# Autodesk Inventor assembly: volledige behuizing
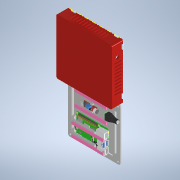
[picture p0: Inventor's stored thumbnail of the model, 180x180]
Saved by Autodesk Inventor 2021 (Build 250183000, 183)
## iProperties
Created: 2023-10-02
Part Number: volledige behuizing
Document SubType Name: Assembly
Designer: Elias
Author: Elias
## Documents named in this file (11)
- D:\Hoge school ICT\2.0 Project experience 2.1\Tekeningen\volledige behuizing.iam
- D:\Hoge school ICT\2.0 Project experience 2.1\Tekeningen\Led behuizing.ipt
- D:\Hoge school ICT\2.0 Project experience 2.1\Tekeningen\Led deksel.ipt
- D:\Hoge school ICT\2.0 Project experience 2.1\Tekeningen\Raspberry Pi 4 Model B.iam
- D:\Hoge school ICT\2.0 Project experience 2.1\Tekeningen\zweef.ipt
- D:\Hoge school ICT\2.0 Project experience 2.1\Tekeningen\geluid sensor.ipt
- D:\Hoge school ICT\2.0 Project experience 2.1\Tekeningen\zweef-01.ipt
- D:\Hoge school ICT\2.0 Project experience 2.1\Tekeningen\koppelstuk.ipt
- D:\Hoge school ICT\2.0 Project experience 2.1\Tekeningen\dc-barrel-jack-adapter-female-with-screw-terminals-1.snapshot.2\dc-barrel-jack-adapter-female.iam
- D:\Hoge school ICT\2.0 Project experience 2.1\Tekeningen\Microphone Module.ipt
- D:\Hoge school ICT\2.0 Project experience 2.1\Tekeningen\ledstrip.ipt
## Components (15 placed, 10 different names)
1. Led behuizing:1 — Mate:2, Mate:3, Mate:4, Flush:6, Mate:9, Flush:7, Mate:12, Flush:10, Tangent:1, Mate:14
2. Led deksel:1 — Mate:2, Mate:3, Insert:1, Insert:2, Mate:4, Flush:1, Mate:5, Flush:2, Mate:6, Mate:8, Flush:4, Flush:5, Tangent:2, Mate:15, Mate:18, Mate:19, Flush:11, Flush:12
3. Raspberry Pi 4 Model B:1 [sub-assembly] — Insert:1, Insert:2
4. zweef:1 — Flush:1, Mate:5, Flush:2, Mate:7, Flush:3, Mate:17
5. geluid sensor:1 — Mate:8, Flush:4, Flush:5
6. zweef-01:1 — Mate:6, Mate:7, Flush:3, Mate:16
7. Led behuizing:2 — Flush:6, Mate:9, Flush:7, Mate:10, Mate:11, Flush:8, Mate:13, Flush:9
8. koppelstuk:1 — Mate:10, Mate:11, Flush:8
9. koppelstuk:2 — Mate:12, Mate:13, Flush:9
10. dc-barrel-jack-adapter-female:1 [sub-assembly] — Flush:10, Tangent:1, Mate:14
11. Microphone Module:2 — Tangent:2, Mate:15
12. ledstrip:1 — Mate:18, Flush:11, Flush:12, Flush:13, Flush:14, Mate:20
13. ledstrip:2 — Mate:19, Flush:13, Mate:20, Mate:21
14. ledstrip:3 — Mate:16, Flush:14, Mate:21, Mate:22, Flush:15
15. ledstrip:4 — Mate:17, Flush:15, Mate:22
## Relationships (40: Mate 21, Flush 15, Insert 2, Tangent 2)
- Mate:2: Led behuizing:1 ↔ Led deksel:1
- Mate:3: Led behuizing:1 ↔ Led deksel:1
- Insert:1: Led deksel:1 ↔ Raspberry Pi 4 Model B:1
- Insert:2: Led deksel:1 ↔ Raspberry Pi 4 Model B:1
- Mate:4: Led behuizing:1 ↔ Led deksel:1
- Flush:1 (20 mm): Led deksel:1 ↔ zweef:1
- Mate:5: Led deksel:1 ↔ zweef:1
- Flush:2 (18 mm): Led deksel:1 ↔ zweef:1
- Mate:6: Led deksel:1 ↔ zweef-01:1
- Mate:7 (20 mm): zweef:1 ↔ zweef-01:1
- Flush:3: zweef:1 ↔ zweef-01:1
- Mate:8: Led deksel:1 ↔ geluid sensor:1
- Flush:4 (20 mm): Led deksel:1 ↔ geluid sensor:1
- Flush:5 (70 mm): Led deksel:1 ↔ geluid sensor:1
- Flush:6: Led behuizing:1 ↔ Led behuizing:2
- Mate:9: Led behuizing:1 ↔ Led behuizing:2
- Flush:7: Led behuizing:1 ↔ Led behuizing:2
- Mate:10: Led behuizing:2 ↔ koppelstuk:1
- Mate:11: Led behuizing:2 ↔ koppelstuk:1
- Flush:8: Led behuizing:2 ↔ koppelstuk:1
- Mate:12: Led behuizing:1 ↔ koppelstuk:2
- Mate:13: Led behuizing:2 ↔ koppelstuk:2
- Flush:9: Led behuizing:2 ↔ koppelstuk:2
- Flush:10 (-30 mm): Led behuizing:1 ↔ dc-barrel-jack-adapter-female:1
- Tangent:1: Led behuizing:1 ↔ dc-barrel-jack-adapter-female:1
- Mate:14 (25 mm): Led behuizing:1 ↔ dc-barrel-jack-adapter-female:1
- Tangent:2: Led deksel:1 ↔ Microphone Module:2
- Mate:15: Led deksel:1 ↔ Microphone Module:2
- Mate:16: zweef-01:1 ↔ ledstrip:3
- Mate:17: zweef:1 ↔ ledstrip:4
- Mate:18: Led deksel:1 ↔ ledstrip:1
- Mate:19: Led deksel:1 ↔ ledstrip:2
- Flush:11 (5 mm): Led deksel:1 ↔ ledstrip:1
- Flush:12 (-5 mm): Led deksel:1 ↔ ledstrip:1
- Flush:13: ledstrip:1 ↔ ledstrip:2
- Flush:14 (-10 mm): ledstrip:1 ↔ ledstrip:3
- Flush:15: ledstrip:3 ↔ ledstrip:4
- Mate:20 (30 mm): ledstrip:1 ↔ ledstrip:2
- Mate:21 (20 mm): ledstrip:2 ↔ ledstrip:3
- Mate:22 (25 mm): ledstrip:3 ↔ ledstrip:4
